# Autodesk Inventor assembly: B
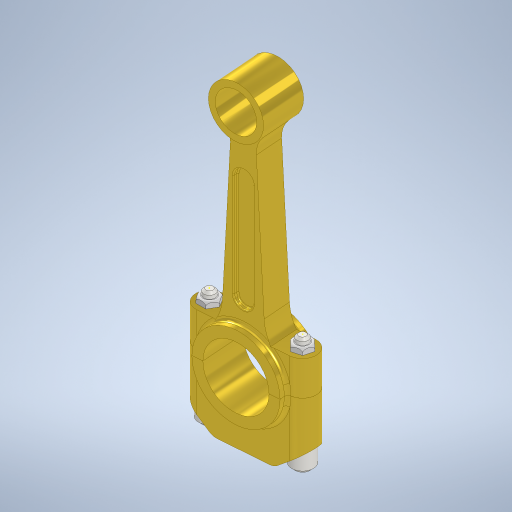
[picture p0: Inventor's stored thumbnail of the model, 512x512]
Saved by Autodesk Inventor 2023 (Build 270158000, 158)
## iProperties
Created: 2025-10-05
Part Number: B
Document SubType Name: Assembly
Designer: ayush
Author: ayush
## Documents named in this file (5)
- C:\Users\ayush\Desktop\INVENTOR FILES COLLEGE\engine\B.iam
- C:\Users\ayush\Desktop\INVENTOR FILES COLLEGE\engine\Part3 CONNECTING ROD.ipt
- C:\Users\ayush\Desktop\INVENTOR FILES COLLEGE\engine\Part4 CONNECTING CAP.ipt
- C:\Users\ayush\Desktop\INVENTOR FILES COLLEGE\engine\BOLT.ipt
- C:\Users\ayush\Desktop\INVENTOR FILES COLLEGE\engine\NUT.ipt
## Components (6 placed, 4 different names)
1. Part3 CONNECTING ROD:1 — Mate:1, Flush:1, Mate:2, Mate:3, Mate:4, Mate:11, Mate:12
2. Part4 CONNECTING CAP:1 — Mate:1, Flush:1, Mate:2, Mate:3, Mate:4, Mate:5, Mate:6, Mate:7, Mate:8
3. BOLT:1 — Mate:5, Mate:8, Mate:9
4. BOLT:2 — Mate:6, Mate:7, Mate:10
5. NUT:1 — Mate:9, Mate:11
6. NUT:2 — Mate:10, Mate:12
## Relationships (13: Mate 12, Flush 1)
- Mate:1: Part3 CONNECTING ROD:1 ↔ Part4 CONNECTING CAP:1
- Flush:1: Part3 CONNECTING ROD:1 ↔ Part4 CONNECTING CAP:1
- Mate:2: Part3 CONNECTING ROD:1 ↔ Part4 CONNECTING CAP:1
- Mate:3: Part3 CONNECTING ROD:1 ↔ Part4 CONNECTING CAP:1
- Mate:4: Part3 CONNECTING ROD:1 ↔ Part4 CONNECTING CAP:1
- Mate:5: Part4 CONNECTING CAP:1 ↔ BOLT:1
- Mate:6: Part4 CONNECTING CAP:1 ↔ BOLT:2
- Mate:7: Part4 CONNECTING CAP:1 ↔ BOLT:2
- Mate:8: Part4 CONNECTING CAP:1 ↔ BOLT:1
- Mate:9: BOLT:1 ↔ NUT:1
- Mate:10: BOLT:2 ↔ NUT:2
- Mate:11: Part3 CONNECTING ROD:1 ↔ NUT:1
- Mate:12: Part3 CONNECTING ROD:1 ↔ NUT:2
